# Autodesk Inventor assembly: rotor-with-sliders
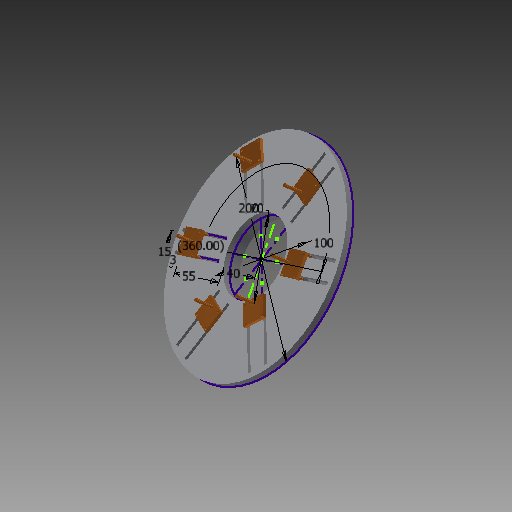
[picture p0: Inventor's stored thumbnail of the model, 512x512]
Saved by Autodesk Inventor 2018 (Build 220112000, 112)
## iProperties
Created: 2024-05-02
Part Number: rotor-with-sliders
Document SubType Name: Assembly
Designer: neo
Author: neo
## Documents named in this file (3)
- D:\projects\kreion\design1\3d\rotor-with-sliders.iam
- D:\projects\kreion\design1\3d\rotor.ipt
- D:\projects\kreion\design1\3d\slider.ipt
## Components (7 placed, 2 different names)
1. rotor:1 — Mate:1, Tangent:1, Tangent:2, Mate:2, Tangent:3, Tangent:4, Tangent:5, Tangent:6, Tangent:7, Tangent:8, Tangent:9, Tangent:10, Tangent:11, Tangent:12
2. slider:1 — Mate:1, Tangent:1, Tangent:2
3. slider:2 — Flush:1, Tangent:11, Tangent:12
4. slider:3 — Flush:1, Flush:2, Tangent:9, Tangent:10
5. slider:4 — Flush:2, Flush:4, Tangent:5, Tangent:6
6. slider:5 — Flush:3, Flush:4, Mate:2, Tangent:7, Tangent:8
7. slider:6 — Flush:3, Tangent:3, Tangent:4
## Relationships (18: Tangent 12, Flush 4, Mate 2)
- Mate:1: rotor:1 ↔ slider:1
- Tangent:1: rotor:1 ↔ slider:1
- Tangent:2: rotor:1 ↔ slider:1
- Flush:1: slider:2 ↔ slider:3
- Flush:2: slider:3 ↔ slider:4
- Flush:3: slider:5 ↔ slider:6
- Flush:4: slider:4 ↔ slider:5
- Mate:2: rotor:1 ↔ slider:5
- Tangent:3: rotor:1 ↔ slider:6
- Tangent:4: rotor:1 ↔ slider:6
- Tangent:5: rotor:1 ↔ slider:4
- Tangent:6: rotor:1 ↔ slider:4
- Tangent:7: rotor:1 ↔ slider:5
- Tangent:8: rotor:1 ↔ slider:5
- Tangent:9: rotor:1 ↔ slider:3
- Tangent:10: rotor:1 ↔ slider:3
- Tangent:11: rotor:1 ↔ slider:2
- Tangent:12: rotor:1 ↔ slider:2
